# Autodesk Inventor assembly: Tension4
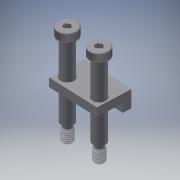
[picture p0: Inventor's stored thumbnail of the model, 180x180]
Saved by Autodesk Inventor 2017 (Build 210142000, 142)
## iProperties
Created: 2018-05-12
Part Number: Tension4
Document SubType Name: Assembly
Designer: User
Author: User
## Documents named in this file (3)
- C:\Robotics\CAD\2018-19_CAD\Offseason\Tension4.iam
- C:\Robotics\CAD\COTSParts\Fasteners\91259A633_ALLOY STEEL SHOULDER SCREW.ipt
- C:\Robotics\CAD\2018-19_CAD\Offseason\TensionerPlate4.ipt
## Components (3 placed, 2 different names)
1. 91259A633_ALLOY STEEL SHOULDER SCREW:1 — Mate:1, Flush:1
2. 91259A633_ALLOY STEEL SHOULDER SCREW:2 — Mate:2, Flush:1
3. TensionerPlate4:1 — Mate:1, Mate:2
## Relationships (3: Mate 2, Flush 1)
- Mate:1: 91259A633_ALLOY STEEL SHOULDER SCREW:1 ↔ TensionerPlate4:1
- Mate:2: 91259A633_ALLOY STEEL SHOULDER SCREW:2 ↔ TensionerPlate4:1
- Flush:1: 91259A633_ALLOY STEEL SHOULDER SCREW:1 ↔ 91259A633_ALLOY STEEL SHOULDER SCREW:2
